# Autodesk Inventor assembly: ALL
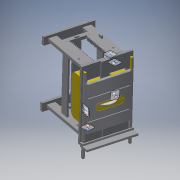
[picture p0: Inventor's stored thumbnail of the model, 180x180]
Saved by Autodesk Inventor 2019.4 (Build 234330000, 330)
## iProperties
Created: 2019-12-14
Part Number: ALL
Document SubType Name: Assembly
Designer: fabfarm
Author: fabfarm
## Documents named in this file (7)
- D:\Users\fabfarm\Documents\Saw table\ALL.iam
- D:\Users\fabfarm\Documents\Saw table\Table_foot.iam
- D:\Users\fabfarm\Documents\Saw table\Table_plate.ipt
- D:\Users\fabfarm\Documents\Saw table\Table_ajutable_part.iam
- D:\Users\fabfarm\Downloads\table-saw-portable-de-walt-1.snapshot.1\TableSaw_Bench3.ipt
- D:\Users\fabfarm\Documents\Saw table\support.ipt
- D:\Users\fabfarm\Documents\Saw table\Jonction.ipt
## Components (12 placed, 6 different names)
1. Table_plate:1 — Mate:7, Mate:8, Mate:9, Mate:10, Flush:17, Flush:18, Flush:24, Flush:25, Mate:25, Flush:26
2. Table_ajutable_part:1 [sub-assembly] — Flush:2, Mate:4, Flush:12, Mate:9, Mate:23
3. Table_ajutable_part:2 [sub-assembly] — Flush:2, Mate:5, Flush:11, Mate:10, Mate:16, Flush:19, Mate:24, Mate:26
4. Table_foot:1 [sub-assembly] — Mate:5, Flush:8, Flush:11, Flush:20, Flush:23, Mate:19
5. Table_foot:2 [sub-assembly] — Mate:4, Flush:8, Flush:12, Mate:17, Flush:22, Mate:20
6. TableSaw_Bench3:1 — Mate:7, Mate:8, Mate:12, Mate:14, Mate:15
7. support:1 — Mate:14, Flush:18, Mate:15, Mate:28
8. support:2 — Mate:12, Flush:17, Mate:27
9. Jonction:1 — Mate:16, Flush:19, Flush:20
10. Jonction:2 — Mate:17, Flush:21, Flush:22, Mate:20
11. Jonction:3 — Flush:21, Flush:23, Mate:19
12. Table_plate:2 — Flush:24, Flush:25, Mate:23, Mate:24, Mate:25, Flush:26, Mate:26, Mate:27, Mate:28
## Relationships (33: Mate 19, Flush 14)
- Flush:2: Table_ajutable_part:1 ↔ Table_ajutable_part:2
- Mate:4: Table_ajutable_part:1 ↔ Table_foot:2
- Mate:5: Table_ajutable_part:2 ↔ Table_foot:1
- Flush:8: Table_foot:1 ↔ Table_foot:2
- Flush:11: Table_ajutable_part:2 ↔ Table_foot:1
- Flush:12: Table_ajutable_part:1 ↔ Table_foot:2
- Mate:7: Table_plate:1 ↔ TableSaw_Bench3:1
- Mate:8: Table_plate:1 ↔ TableSaw_Bench3:1
- Mate:9: Table_plate:1 ↔ Table_ajutable_part:1
- Mate:10: Table_plate:1 ↔ Table_ajutable_part:2
- Mate:12: TableSaw_Bench3:1 ↔ support:2
- Flush:17: Table_plate:1 ↔ support:2
- Mate:14: TableSaw_Bench3:1 ↔ support:1
- Flush:18: Table_plate:1 ↔ support:1
- Mate:15: TableSaw_Bench3:1 ↔ support:1
- Mate:16: Table_ajutable_part:2 ↔ Jonction:1
- Flush:19 (-20 mm): Table_ajutable_part:2 ↔ Jonction:1
- Flush:20 (200 mm): Table_foot:1 ↔ Jonction:1
- Mate:17: Table_foot:2 ↔ Jonction:2
- Flush:21: Jonction:2 ↔ Jonction:3
- Flush:22 (40 mm): Table_foot:2 ↔ Jonction:2
- Flush:23 (40 mm): Table_foot:1 ↔ Jonction:3
- Mate:19: Table_foot:1 ↔ Jonction:3
- Mate:20 (200 mm): Table_foot:2 ↔ Jonction:2
- Flush:24: Table_plate:1 ↔ Table_plate:2
- Flush:25: Table_plate:1 ↔ Table_plate:2
- Mate:23: Table_ajutable_part:1 ↔ Table_plate:2
- Mate:24: Table_ajutable_part:2 ↔ Table_plate:2
- Mate:25: Table_plate:1 ↔ Table_plate:2
- Flush:26: Table_plate:1 ↔ Table_plate:2
- Mate:26: Table_ajutable_part:2 ↔ Table_plate:2
- Mate:27: support:2 ↔ Table_plate:2
- Mate:28: support:1 ↔ Table_plate:2
